# Autodesk Inventor assembly: PhoneCordHolder
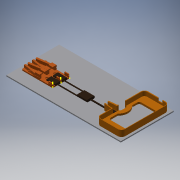
[picture p0: Inventor's stored thumbnail of the model, 180x180]
Saved by Autodesk Inventor 2017 (Build 210142000, 142)
## iProperties
Created: 2017-12-02
Part Number: PhoneCordHolder
Document SubType Name: Assembly
Designer: User
Author: User
## Documents named in this file (5)
- C:\Robotics\CAD\2017-18_CAD\PhoneCordHolder.iam
- C:\Robotics\CAD\2017-18_CAD\phone holder base.ipt
- C:\Robotics\CAD\2017-18_CAD\Phone_Case_Driver.ipt
- C:\Robotics\CAD\2017-18_CAD\phone wire.ipt
- C:\Robotics\CAD\2017-18_CAD\cord holders ipt.ipt
## Components (5 placed, 4 different names)
1. phone holder base:1 — Mate:1, Flush:1, Flush:2, Mate:2, Mate:4, Mate:6
2. Phone_Case_Driver:1 — Mate:1, Flush:1, Flush:2, Flush:3, Mate:3
3. phone wire:1 — Mate:2, Flush:3, Mate:3, Flush:4, Flush:5, Mate:7, Mate:8
4. cord holders ipt:1 — Mate:4, Flush:5, Mate:8
5. cord holders ipt:2 — Mate:6, Flush:4, Mate:7
## Relationships (12: Mate 7, Flush 5)
- Mate:1: phone holder base:1 ↔ Phone_Case_Driver:1
- Flush:1 (6.35 mm): phone holder base:1 ↔ Phone_Case_Driver:1
- Flush:2 (6.35 mm): phone holder base:1 ↔ Phone_Case_Driver:1
- Mate:2: phone holder base:1 ↔ phone wire:1
- Flush:3: Phone_Case_Driver:1 ↔ phone wire:1
- Mate:3: Phone_Case_Driver:1 ↔ phone wire:1
- Mate:4: phone holder base:1 ↔ cord holders ipt:1
- Mate:6: phone holder base:1 ↔ cord holders ipt:2
- Flush:4: phone wire:1 ↔ cord holders ipt:2
- Flush:5: phone wire:1 ↔ cord holders ipt:1
- Mate:7: phone wire:1 ↔ cord holders ipt:2
- Mate:8: phone wire:1 ↔ cord holders ipt:1
